# Autodesk Inventor assembly: Shooter-pipes
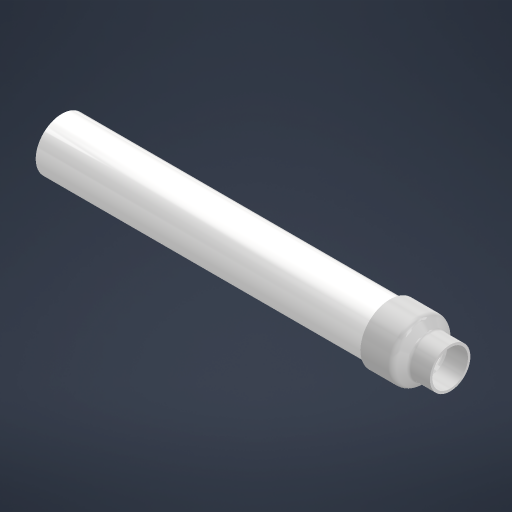
[picture p0: Inventor's stored thumbnail of the model, 512x512]
Saved by Autodesk Inventor 2023 (Build 270158000, 158)
## iProperties
Created: 2022-06-22
Part Number: Shooter-pipes
Document SubType Name: Assembly
Designer: timmy
Author: timmy
## Documents named in this file (3)
- R:\Inventor\RoboCatz\T-Shirt\Rev2-Better\Shooter-pipes.iam
- R:\Inventor\RoboCatz\T-Shirt\Rev2-Better\pvc-pipe-fittings-1.snapshot.2\3x2_R-Socket.ipt
- R:\Inventor\RoboCatz\T-Shirt\Rev2-Better\Shooter-pipes.ipt
## Components (2 placed, 2 different names)
1. 3x2_R-Socket:1 — Mate:1, Mate:2
2. Shooter-pipes:1 — Mate:1, Mate:2
## Relationships (2: Mate 2)
- Mate:1: 3x2_R-Socket:1 ↔ Shooter-pipes:1
- Mate:2: 3x2_R-Socket:1 ↔ Shooter-pipes:1
